# Autodesk Inventor assembly: am-940a-6-HiGrip-_MIR
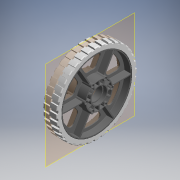
[picture p0: Inventor's stored thumbnail of the model, 180x180]
Saved by Autodesk Inventor 2016 SP1 (Build 200210100, 210)
## iProperties
Created: 2014-03-19
Part Number: am-940a-6-HiGrip-_MIR
Description: STEP AP214
Document SubType Name: Assembly
Designer: steele
Title: 6-HiGrip-am-940aSTEP.STEP
Revision Number: ANY
Sending System: SolidWorks 2010
Preprocessor: SwSTEP 2.0
## Documents named in this file (3)
- C:\snobotics\CAD-Development\robSteele\SnoBotics2016\2016-01-23-BallShooter\am-940a-6-HiGrip-_MIR.iam
- C:\snobotics\CAD-Development\robSteele\SnoBotics2016\2016-01-23-BallShooter\6 wheel Rev 4_MIR.ipt
- C:\snobotics\CAD-Development\robSteele\SnoBotics2016\2016-01-23-BallShooter\6 wheel tread II_MIR.ipt
## Components (2 placed, 2 different names)
1. 6 wheel Rev 4_MIR:1
2. 6 wheel tread II_MIR:1 — Flush:1
## Relationships (1: Flush 1)
- Flush:1 (-12.7 mm): 6 wheel tread II_MIR:1
